# Autodesk Inventor assembly: COXA_UNIT_ASM
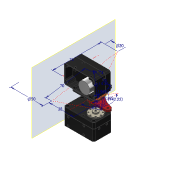
[picture p0: Inventor's stored thumbnail of the model, 180x180]
Saved by Autodesk Inventor 2019.4 (Build 234330000, 330)
## iProperties
Created: 2019-10-21
Part Number: COXA_UNIT_ASM
Material: 一般
Document SubType Name: Assembly
Designer: y6tada
Author: y6tada
## Documents named in this file (5)
- C:\Workspace\Yuni8\Asm\COXA_UNIT\COXA_UNIT_ASM.iam
- C:\Workspace\Yuni8\Libs\DYNAMIXEL\XM430\XM430_ASM_WITHOUT-BACK.iam
- C:\Workspace\Yuni8\Asm\COXA_UNIT\COXA_YAW_SERVO_BASE.ipt
- C:\Workspace\Yuni8\Asm\COXA_UNIT\COXA_YAW_SUPPORT-LINK_BACK.ipt
- C:\Workspace\Yuni8\Asm\COXA_UNIT\COXA_ROLL_SERVO-OUTPUT.ipt
## Components (5 placed, 4 different names)
1. XM430_ASM_WITHOUT-BACK:1 [sub-assembly] — メイト:1, メイト:2, メイト:3, メイト:4, 角度:2, メイト:10
2. XM430_ASM_WITHOUT-BACK:2 [sub-assembly] — メイト:7, 角度:2
3. COXA_YAW_SERVO_BASE:1 — メイト:3, メイト:4, フラッシュ:1, メイト:6, メイト:8, メイト:10, メイト:11
4. COXA_YAW_SUPPORT-LINK_BACK:1 — メイト:8, メイト:11, メイト:13, メイト:14
5. COXA_ROLL_SERVO-OUTPUT:1 — メイト:12, メイト:13, メイト:14
## Relationships (15: Mate 12, Angle 2, Flush 1)
- メイト:1 [Mate] (25 mm): XM430_ASM_WITHOUT-BACK:1
- メイト:2 [Mate]: XM430_ASM_WITHOUT-BACK:1
- メイト:3 [Mate]: XM430_ASM_WITHOUT-BACK:1 ↔ COXA_YAW_SERVO_BASE:1
- メイト:4 [Mate]: XM430_ASM_WITHOUT-BACK:1 ↔ COXA_YAW_SERVO_BASE:1
- フラッシュ:1 [Flush]: COXA_YAW_SERVO_BASE:1
- メイト:6 [Mate]: COXA_YAW_SERVO_BASE:1
- 角度:1 [Angle] (0 deg)
- メイト:7 [Mate]: XM430_ASM_WITHOUT-BACK:2
- 角度:2 [Angle] (0 deg): XM430_ASM_WITHOUT-BACK:1 ↔ XM430_ASM_WITHOUT-BACK:2
- メイト:8 [Mate]: COXA_YAW_SERVO_BASE:1 ↔ COXA_YAW_SUPPORT-LINK_BACK:1
- メイト:10 [Mate]: XM430_ASM_WITHOUT-BACK:1 ↔ COXA_YAW_SERVO_BASE:1
- メイト:11 [Mate]: COXA_YAW_SERVO_BASE:1 ↔ COXA_YAW_SUPPORT-LINK_BACK:1
- メイト:12 [Mate]: COXA_ROLL_SERVO-OUTPUT:1
- メイト:13 [Mate]: COXA_YAW_SUPPORT-LINK_BACK:1 ↔ COXA_ROLL_SERVO-OUTPUT:1
- メイト:14 [Mate]: COXA_YAW_SUPPORT-LINK_BACK:1 ↔ COXA_ROLL_SERVO-OUTPUT:1
